# Autodesk Inventor assembly: Arm_bolt_set_2_5_8 x 6
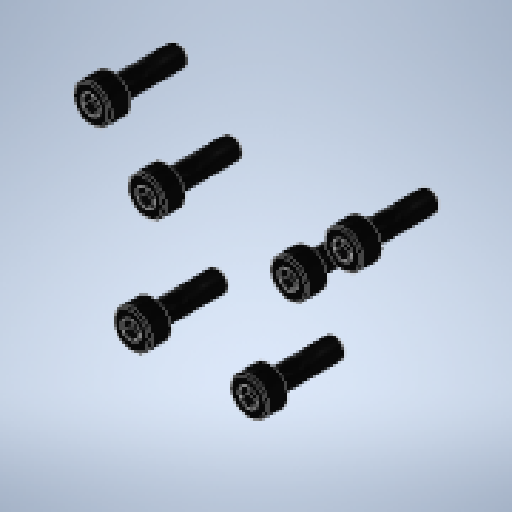
[picture p0: Inventor's stored thumbnail of the model, 512x512]
Saved by Autodesk Inventor 2024 (Build 280153000, 153)
## iProperties
Created: 2024-09-18
Part Number: Arm_bolt_set_2_5_8 x 6
Document SubType Name: Assembly
Designer: Eungang
Author: Eungang
## Documents named in this file (3)
- C:\Users\Eungang\Documents\Inventor\FIGHTING_ROBOT_FINAL\부품\Bolt_Washer_Nut\Arm_bolt_set_2_5_8 x 6.iam
- C:\Users\Eungang\Documents\Inventor\FIGHTING_ROBOT_FINAL\부품\Bolt_Washer_Nut\CSH-ST-M2_5-8_203.ipt
- C:\Users\Eungang\Documents\Inventor\FIGHTING_ROBOT_FINAL\부품\Right_Arm\arm_motor_connecter_bridge.ipt
## Components (7 placed, 2 different names)
1. CSH-ST-M2_5-8_203:1
2. CSH-ST-M2_5-8_203:4 — 삽입:1
3. CSH-ST-M2_5-8_203:5 — 삽입:2
4. CSH-ST-M2_5-8_203:6
5. arm_motor_connecter_bridge:1 — 삽입:1, 삽입:2, 삽입:3, 삽입:4
6. CSH-ST-M2_5-8_203:7 — 삽입:4
7. CSH-ST-M2_5-8_203:8 — 삽입:3
## Relationships (4: Insert 4)
- 삽입:1 [Insert]: CSH-ST-M2_5-8_203:4 ↔ arm_motor_connecter_bridge:1
- 삽입:2 [Insert]: CSH-ST-M2_5-8_203:5 ↔ arm_motor_connecter_bridge:1
- 삽입:3 [Insert]: arm_motor_connecter_bridge:1 ↔ CSH-ST-M2_5-8_203:8
- 삽입:4 [Insert]: arm_motor_connecter_bridge:1 ↔ CSH-ST-M2_5-8_203:7
